# Autodesk Inventor assembly: PCB Component
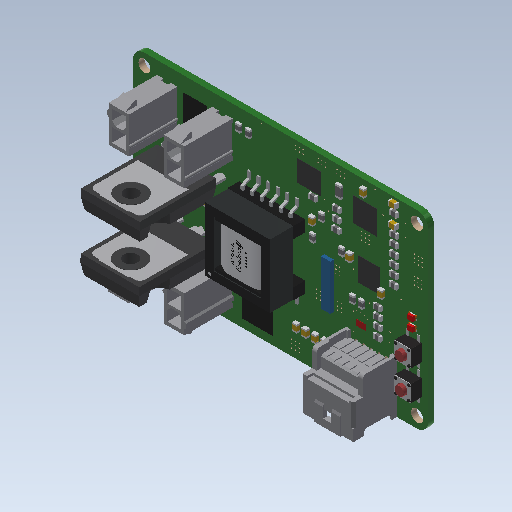
[picture p0: Inventor's stored thumbnail of the model, 512x512]
Saved by Autodesk Inventor 2020 (Build 240168000, 168)
## iProperties
Created: 2019-05-25
Part Number: PCB Component
Document SubType Name: Assembly
Designer: jg_ma
Author: jg_ma
## Documents named in this file (16)
- C:\Users\Acer\Documents\ssl-mechanics\V2.1(LARC2019)\Inventor\sec_floor\Components\KickerBoard\PCB Component.iam
- C:\Users\Acer\Documents\ssl-mechanics\V2.1(LARC2019)\Inventor\sec_floor\Components\KickerBoard\Board.ipt
- C:\Users\Acer\Documents\ssl-mechanics\V2.1(LARC2019)\Inventor\sec_floor\Components\KickerBoard\C0805K.ipt
- C:\Users\Acer\Documents\ssl-mechanics\V2.1(LARC2019)\Inventor\sec_floor\Components\KickerBoard\153CLV-1010.ipt
- C:\Users\Acer\Documents\ssl-mechanics\V2.1(LARC2019)\Inventor\sec_floor\Components\KickerBoard\SMC.ipt
- C:\Users\Acer\Documents\ssl-mechanics\V2.1(LARC2019)\Inventor\sec_floor\Components\KickerBoard\SOIC8.ipt
- C:\Users\Acer\Documents\ssl-mechanics\V2.1(LARC2019)\Inventor\sec_floor\Components\KickerBoard\TSSOP20P.ipt
- C:\Users\Acer\Documents\ssl-mechanics\V2.1(LARC2019)\Inventor\sec_floor\Components\KickerBoard\CHIP-LED0805.ipt
- C:\Users\Acer\Documents\ssl-mechanics\V2.1(LARC2019)\Inventor\sec_floor\Components\KickerBoard\R0805.ipt
- C:\Users\Acer\Documents\ssl-mechanics\V2.1(LARC2019)\Inventor\sec_floor\Components\KickerBoard\R1206.ipt
- C:\Users\Acer\Documents\ssl-mechanics\V2.1(LARC2019)\Inventor\sec_floor\Components\KickerBoard\QFN25X15.ipt
- C:\Users\Acer\Documents\ssl-mechanics\V2.1(LARC2019)\Inventor\sec_floor\Components\KickerBoard\55959-1030_stp\559591030.ipt
- C:\Users\Acer\Documents\ssl-mechanics\V2.1(LARC2019)\Inventor\sec_floor\Components\KickerBoard\Infineon-STP_PG-TO247-3-901-P-v01_00-EN\Infineon-STP_PG-TO247-3-901-P-v01_00-EN.iam
- C:\Users\Acer\Documents\ssl-mechanics\V2.1(LARC2019)\Inventor\sec_floor\Components\KickerBoard\Coilcraft-DA2033-AL\Coilcraft-DA2033-AL.ipt
- C:\Users\Acer\Documents\ssl-mechanics\V2.1(LARC2019)\Inventor\sec_floor\Components\KickerBoard\39-28-1023_stp\039281023.ipt
- C:\Users\Acer\Documents\ssl-mechanics\V2.1(LARC2019)\Inventor\sec_floor\Components\KickerBoard\tactile-switches-smd-1.snapshot.7\Tact Switch SMD 4.5x4.5mm.ipt
## Components (59 placed, 54 different names)
1. Board:1 — Mate:1, Flush:1, Flush:2, Flush:3, Flush:4, Mate:2, Mate:3, Mate:4, Mate:5, Mate:6, Mate:7, Mate:8, Mate:9, Flush:5, Flush:6, Flush:7, Flush:8, Flush:9, Mate:10, Mate:11, Flush:10
2. C0805K:C1
3. C0805K:C12
4. C0805K:C13
5. C0805K:C14
6. C0805K:C18
7. C0805K:C19
8. C0805K:C20
9. C0805K:C21
10. C0805K:C22
11. C0805K:C23
12. C0805K:C24
13. C0805K:C25
14. 153CLV-1010:C57
15. SMC:D1
16. SMC:D2
17. SMC:D3
18. SOIC8:IC10
19. SOIC8:IC8
20. SOIC8:Q1
21. TSSOP20P:IC9
22. CHIP-LED0805:+50V
23. CHIP-LED0805:3V3
24. R0805:R1
25. R0805:R10
26. R0805:R11
27. R0805:R13
28. R0805:R14
29. R0805:R15
30. R0805:R16
31. R0805:R18
32. R0805:R19
33. R0805:R2
34. R0805:R21
35. R0805:R22R
36. R0805:R29
37. R0805:R3
38. R0805:R4
39. R0805:R5
40. R0805:R6
41. R0805:R8
42. R0805:R9
43. R0805:R28
44. R0805:R7
45. R0805:R12
46. R0805:R17
47. R0805:R22
48. R1206:R20
49. QFN25X15:E1
50. 559591030:1 — Mate:1, Flush:1, Flush:2
51. Infineon-STP_PG-TO247-3-901-P-v01_00-EN:1 [sub-assembly] — Flush:3, Mate:3
52. Infineon-STP_PG-TO247-3-901-P-v01_00-EN:2 [sub-assembly] — Flush:4, Mate:2
53. Coilcraft-DA2033-AL:1 — Mate:4, Mate:5
54. 039281023:1 — Mate:6, Flush:5
55. 039281023:2 — Mate:8, Flush:8
56. 039281023:3 — Mate:9, Flush:7
57. 039281023:4 — Mate:7, Flush:6
58. Tact Switch SMD 4.5x4.5mm:1 — Flush:9, Mate:10
59. Tact Switch SMD 4.5x4.5mm:2 — Mate:11, Flush:10
## Relationships (21: Mate 11, Flush 10)
- Mate:1: Board:1 ↔ 559591030:1
- Flush:1: Board:1 ↔ 559591030:1
- Flush:2 (8.3 mm): Board:1 ↔ 559591030:1
- Flush:3 (14.8 mm): Board:1 ↔ Infineon-STP_PG-TO247-3-901-P-v01_00-EN:1
- Flush:4 (29.8 mm): Board:1 ↔ Infineon-STP_PG-TO247-3-901-P-v01_00-EN:2
- Mate:2: Board:1 ↔ Infineon-STP_PG-TO247-3-901-P-v01_00-EN:2
- Mate:3: Board:1 ↔ Infineon-STP_PG-TO247-3-901-P-v01_00-EN:1
- Mate:4: Board:1 ↔ Coilcraft-DA2033-AL:1
- Mate:5 (16.5 mm): Board:1 ↔ Coilcraft-DA2033-AL:1
- Mate:6: Board:1 ↔ 039281023:1
- Mate:7: Board:1 ↔ 039281023:4
- Mate:8: Board:1 ↔ 039281023:2
- Mate:9: Board:1 ↔ 039281023:3
- Flush:5 (3.4 mm): Board:1 ↔ 039281023:1
- Flush:6 (3.4 mm): Board:1 ↔ 039281023:4
- Flush:7 (3.4 mm): Board:1 ↔ 039281023:3
- Flush:8 (3.4 mm): Board:1 ↔ 039281023:2
- Flush:9 (1.7 mm): Board:1 ↔ Tact Switch SMD 4.5x4.5mm:1
- Mate:10: Board:1 ↔ Tact Switch SMD 4.5x4.5mm:1
- Mate:11: Board:1 ↔ Tact Switch SMD 4.5x4.5mm:2
- Flush:10 (1.7 mm): Board:1 ↔ Tact Switch SMD 4.5x4.5mm:2
